# Autodesk Inventor assembly: Assembly1
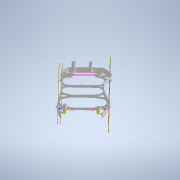
[picture p0: Inventor's stored thumbnail of the model, 180x180]
Saved by Autodesk Inventor 2020.3 (Build 243373000, 373)
## iProperties
Created: 2020-09-10
Part Number: Assembly1
Document SubType Name: Assembly
Designer: Mara
Author: Mara
## Documents named in this file (3)
- C:\Users\Mara\Masterarbeit_CAD\Schuh\Schuh_Kombi_sg.iam
- C:\Users\Mara\Masterarbeit_CAD\Schuh\Schuh_Befestigung_sg.ipt
- C:\Users\Mara\Masterarbeit_CAD\Schuh\Schuh_mit_Halterungsbereich.ipt
## Components (2 placed, 2 different names)
1. Schuh_Befestigung_sg:1 — Flush:1, Mate:1
2. Schuh_mit_Halterungsbereich:1 — Flush:1, Mate:1
## Relationships (2: Flush 1, Mate 1)
- Flush:1 (6 mm): Schuh_Befestigung_sg:1 ↔ Schuh_mit_Halterungsbereich:1
- Mate:1 (-1 mm): Schuh_Befestigung_sg:1 ↔ Schuh_mit_Halterungsbereich:1
